# Autodesk Inventor assembly: ADSK-MH-10000
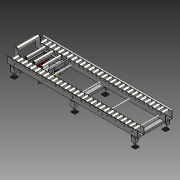
[picture p0: Inventor's stored thumbnail of the model, 180x180]
Saved by Autodesk Inventor 2014 (Build 180170000, 170)
## iProperties
Created: 2013-08-01
Part Number: ADSK-MH-10000
Document SubType Name: Assembly
Designer: Demir Ali
Description: Overall Conveyor Assembly
Engineer: Demir Ali
Checked By: Demir Ali
RuleStatus: InUse
Company: Autodesk Ltd
Author: Demir Ali
Keywords: Roller Conveyor
Revision Number: A
## Documents named in this file (10)
- D:\Vault Workspace\Design Data\Projects\Discharge Conveyor\ADSK-MH-10000.iam
- D:\Vault Workspace\Design Data\Projects\Discharge Conveyor\ADSK-MH-10003.ipt
- D:\Vault Workspace\Design Data\Projects\Discharge Conveyor\ADSK-MH-10007.ipt
- D:\Vault Workspace\Design Data\Projects\Discharge Conveyor\ADSK-MH-10009.ipt
- D:\Vault Workspace\Design Data\Projects\Discharge Conveyor\ADSK-MH-10010.iam
- D:\Vault Workspace\Design Data\Projects\Discharge Conveyor\ADSK-MH-10013.ipt
- D:\Vault Workspace\Design Data\Projects\Discharge Conveyor\ADSK-MH-10014.iam
- D:\Vault Workspace\Design Data\Projects\Discharge Conveyor\ADSK-MH-10018.ipt
- D:\Vault Workspace\Design Data\Projects\Discharge Conveyor\ADSK-MH-10019.iam
- D:\Vault Workspace\Design Data\Projects\Discharge Conveyor\ADSK-MH-10027.iam
## Components (82 placed, 12 different names)
1. Outer Beam Plate — Flush:4, Mate:6, Mate:7, Angle:3, Mate:10, Mate:11, Insert:16, Insert:18, Flush:7, Flush:8, Flush:9, Flush:10
2. ADSK-MH-10003:2 — Flush:5, Mate:8, Mate:9, Mate:13, Mate:17, Mate:18
3. Inner Beam Plate A — Flush:4, Mate:6, Mate:7, Insert:21, Mate:15
4. Inner Beam Plate B — Flush:5, Mate:8, Mate:9
5. Top_Roller_assem [sub-assembly] — Insert:21
6. Discharge_assem [sub-assembly] — Mate:18, Flush:6, Flush:10
7. ADSK-MH-10010:1 [sub-assembly] — Angle:3, Mate:10, Mate:11, Flush:6
8. ADSK-MH-10010:2 [sub-assembly]
9. ADSK-MH-10010:3 [sub-assembly]
10. Support_beam_spacer — Mate:14, Mate:17
11. ADSK-MH-10013:2 — Insert:16, Mate:14, Mate:16
12. Support_bar_long — Mate:15, Mate:16
13. ADSK-MH-10013:4
14. ADSK-MH-10013:5
15. ADSK-MH-10018:3
16. ADSK-MH-10013:6
17. ADSK-MH-10013:7
18. ADSK-MH-10018:4
19. ADSK-MH-10013:8
20. ADSK-MH-10013:9
21. ADSK-MH-10018:5
22. ADSK-MH-10013:10
23. ADSK-MH-10013:11
24. ADSK-MH-10018:6
25. ADSK-MH-10014:2 [sub-assembly] — Mate:12, Mate:13
26. ADSK-MH-10014:1 [sub-assembly] — Insert:18, Mate:12
27. ADSK-MH-10014:3 [sub-assembly]
28. ADSK-MH-10014:4 [sub-assembly]
29. ADSK-MH-10014:5 [sub-assembly]
30. ADSK-MH-10014:6 [sub-assembly]
31. ADSK-MH-10014:7 [sub-assembly]
32. ADSK-MH-10014:8 [sub-assembly]
33. ADSK-MH-10014:9 [sub-assembly]
34. ADSK-MH-10014:10 [sub-assembly]
35. ADSK-MH-10014:11 [sub-assembly]
36. ADSK-MH-10014:12 [sub-assembly]
37. ADSK-MH-10014:13 [sub-assembly]
38. ADSK-MH-10014:14 [sub-assembly]
39. ADSK-MH-10014:15 [sub-assembly]
40. ADSK-MH-10014:16 [sub-assembly]
41. ADSK-MH-10014:17 [sub-assembly]
42. ADSK-MH-10014:18 [sub-assembly]
43. ADSK-MH-10014:19 [sub-assembly]
44. ADSK-MH-10014:20 [sub-assembly]
45. ADSK-MH-10014:21 [sub-assembly]
46. ADSK-MH-10014:22 [sub-assembly]
47. ADSK-MH-10014:23 [sub-assembly]
48. ADSK-MH-10014:24 [sub-assembly]
49. ADSK-MH-10014:25 [sub-assembly]
50. ADSK-MH-10014:26 [sub-assembly]
51. ADSK-MH-10014:27 [sub-assembly]
52. ADSK-MH-10014:28 [sub-assembly]
53. ADSK-MH-10014:29 [sub-assembly]
54. ADSK-MH-10014:30 [sub-assembly]
55. ADSK-MH-10014:31 [sub-assembly]
56. ADSK-MH-10014:32 [sub-assembly]
57. ADSK-MH-10014:33 [sub-assembly]
58. ADSK-MH-10014:34 [sub-assembly]
59. ADSK-MH-10014:35 [sub-assembly]
60. ADSK-MH-10014:36 [sub-assembly]
61. ADSK-MH-10014:37 [sub-assembly]
62. ADSK-MH-10014:38 [sub-assembly]
63. ADSK-MH-10014:39 [sub-assembly]
64. ADSK-MH-10014:40 [sub-assembly]
65. ADSK-MH-10014:41 [sub-assembly]
66. ADSK-MH-10014:42 [sub-assembly]
67. ADSK-MH-10014:43 [sub-assembly]
68. ADSK-MH-10014:44 [sub-assembly]
69. ADSK-MH-10014:45 [sub-assembly]
70. ADSK-MH-10014:46 [sub-assembly]
71. ADSK-MH-10014:47 [sub-assembly]
72. ADSK-MH-10014:48 [sub-assembly]
73. ADSK-MH-10014:49 [sub-assembly]
74. ADSK-MH-10014:50 [sub-assembly]
75. ADSK-MH-10014:51 [sub-assembly]
76. ADSK-MH-10014:52 [sub-assembly]
77. ADSK-MH-10014:53 [sub-assembly]
78. ADSK-MH-10014:54 [sub-assembly]
79. ADSK-MH-10014:55 [sub-assembly]
80. ADSK-MH-10014:56 [sub-assembly]
81. ADSK-MH-10014:57 [sub-assembly]
82. ADSK-MH-10014:58 [sub-assembly]
## Component patterns: (3 elements, first: ADSK-MH-10010:1), (5 elements, first: Support_beam_spacer + ADSK-MH-10013:2 + Support_bar_long), (29 elements, first: ADSK-MH-10014:2 + ADSK-MH-10014:1)
## Relationships (27: Mate 15, Flush 8, Insert 3, Angle 1)
- [Mate]: Outer Beam Plate ↔ ADSK-MH-10003:2
- [Flush]: Outer Beam Plate ↔ ADSK-MH-10003:2
- [Mate] (800 mm): Outer Beam Plate ↔ ADSK-MH-10003:2
- Flush:4: Outer Beam Plate ↔ Inner Beam Plate A
- Mate:6 (150 mm): Outer Beam Plate ↔ Inner Beam Plate A
- Mate:7: Outer Beam Plate ↔ Inner Beam Plate A
- Flush:5: ADSK-MH-10003:2 ↔ Inner Beam Plate B
- Mate:8 (150 mm): ADSK-MH-10003:2 ↔ Inner Beam Plate B
- Mate:9: ADSK-MH-10003:2 ↔ Inner Beam Plate B
- Angle:3 (180 deg): Outer Beam Plate ↔ ADSK-MH-10010:1
- Mate:10: Outer Beam Plate ↔ ADSK-MH-10010:1
- Mate:11: Outer Beam Plate ↔ ADSK-MH-10010:1
- Insert:16: Outer Beam Plate ↔ ADSK-MH-10013:2
- Insert:18: Outer Beam Plate ↔ ADSK-MH-10014:1
- Insert:21: Inner Beam Plate A ↔ Top_Roller_assem
- Mate:12: ADSK-MH-10014:2 ↔ ADSK-MH-10014:1
- Mate:13: ADSK-MH-10003:2 ↔ ADSK-MH-10014:2
- Mate:14: Support_beam_spacer ↔ ADSK-MH-10013:2
- Mate:15: Inner Beam Plate A ↔ Support_bar_long
- Mate:16: ADSK-MH-10013:2 ↔ Support_bar_long
- Mate:17: ADSK-MH-10003:2 ↔ Support_beam_spacer
- Mate:18: ADSK-MH-10003:2 ↔ Discharge_assem
- Flush:6: Discharge_assem ↔ ADSK-MH-10010:1
- Flush:7 (240 mm): Outer Beam Plate
- Flush:8 (-400 mm): Outer Beam Plate
- Flush:9: Outer Beam Plate
- Flush:10 (1000 mm): Outer Beam Plate ↔ Discharge_assem
